# Autodesk Inventor assembly: Push cart wheel assembly
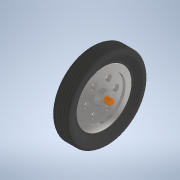
[picture p0: Inventor's stored thumbnail of the model, 180x180]
Saved by Autodesk Inventor 2021 (Build 250183000, 183)
## iProperties
Created: 2022-05-13
Part Number: Push cart wheel assembly
Document SubType Name: Assembly
Designer: kajet
Author: kajet
## Documents named in this file (4)
- C:\Users\kajet\Desktop\HW\SEMESTR 6\PM\Koło_jezdne\Push cart wheel assembly.iam
- C:\Users\kajet\Desktop\HW\SEMESTR 6\PM\Koło_jezdne\Shaft1.ipt
- C:\Users\kajet\Desktop\HW\SEMESTR 6\PM\Koło_jezdne\felga.ipt
- C:\Users\kajet\Desktop\HW\SEMESTR 6\PM\Koło_jezdne\opona.ipt
## Components (3 placed, 3 different names)
1. Shaft:1 — Mate:1, Mate:2, Flush:1, Mate:6, Mate:8
2. felga:1 — Mate:3, Mate:4, Flush:2, Mate:5, Mate:8
3. opona:1 — Mate:3, Mate:4, Flush:2
## Relationships (10: Mate 8, Flush 2)
- Mate:1: Shaft:1
- Mate:2: Shaft:1
- Flush:1: Shaft:1
- Mate:3: felga:1 ↔ opona:1
- Mate:4: felga:1 ↔ opona:1
- Flush:2: felga:1 ↔ opona:1
- Mate:5: felga:1
- Mate:6: Shaft:1
- Mate:7
- Mate:8: Shaft:1 ↔ felga:1
